# Autodesk Inventor assembly: celestronTripodAdapterAssembly
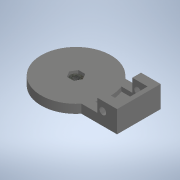
[picture p0: Inventor's stored thumbnail of the model, 180x180]
Saved by Autodesk Inventor 2021.1 (Build 251245000, 245)
## iProperties
Created: 2020-07-29
Part Number: celestronTripodAdapterAssembly
Document SubType Name: Assembly
Designer: robst
Author: robst
## Documents named in this file (3)
- C:\git\CAD-Development\robSteele\ShapeWays\TelescopeProjects\TelescopeMount\celestronTripodAdapterAssembly.iam
- C:\git\CAD-Development\robSteele\ShapeWays\TelescopeProjects\TelescopeMount\celestronTripodAdapter.ipt
- C:\Users\robst\Documents\Inventor\Content Center Files\R2021\en-US\BS EN 24034\ISO 4034 - M10BS EN.ipt
## Components (2 placed, 2 different names)
1. celestronTripodAdapter:1 — Insert:1
2. BS EN 24034 - Metric M10:1 — Insert:1
## Relationships (1: Insert 1)
- Insert:1: celestronTripodAdapter:1 ↔ BS EN 24034 - Metric M10:1
